# Autodesk Inventor assembly: cwiczenie2
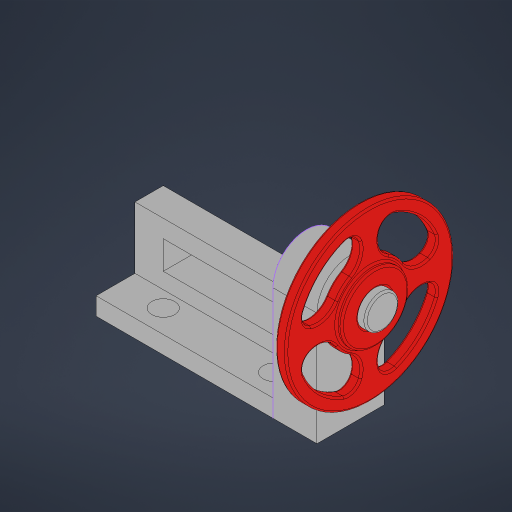
[picture p0: Inventor's stored thumbnail of the model, 512x512]
Saved by Autodesk Inventor 2024 (Build 280153000, 153)
## iProperties
Created: 2024-03-07
Part Number: cwiczenie2
Document SubType Name: Assembly
Designer: Papryk
Author: Papryk
## Documents named in this file (3)
- J:\cwiczenie2.iam
- J:\Part4.ipt
- J:\Part5.ipt
## Components (2 placed, 2 different names)
1. Part4:1 — Mate:1, Mate:2, Mate:3
2. Part5:1 — Mate:1, Mate:2, Mate:3
## Relationships (3: Mate 3)
- Mate:1: Part4:1 ↔ Part5:1
- Mate:2: Part4:1 ↔ Part5:1
- Mate:3: Part4:1 ↔ Part5:1
